# Autodesk Inventor assembly: SMALLER
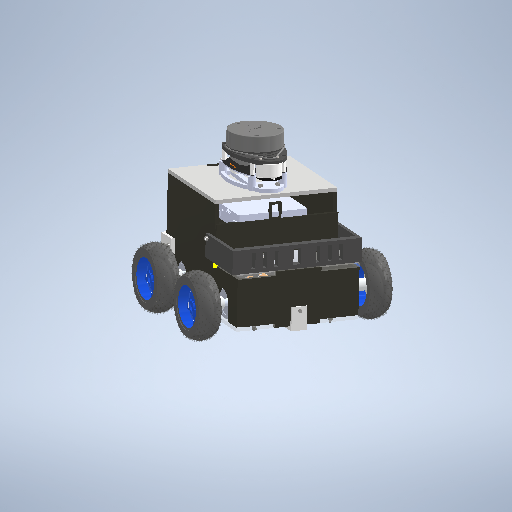
[picture p0: Inventor's stored thumbnail of the model, 512x512]
Saved by Autodesk Inventor 2025.3 (Build 293356030, 356C)
## iProperties
Created: 2026-06-30
Part Number: SMALLER
Document SubType Name: Assembly
Designer: user
Author: user
## Documents named in this file (14)
- C:\Docs\shcool\dojo\CAD_stuff\Final\SMALLER.iam
- C:\Docs\shcool\dojo\CAD_stuff\Final\WHEEL_BASE.iam
- C:\Docs\shcool\dojo\CAD_stuff\Final\back.ipt
- C:\Docs\shcool\dojo\CAD_stuff\Final\Fastener.ipt
- C:\Docs\shcool\dojo\CAD_stuff\Final\SIDE_1.ipt
- C:\Docs\shcool\dojo\CAD_stuff\Final\HOOD_1.ipt
- C:\Docs\shcool\dojo\CAD_stuff\Final\TOP_1.ipt
- C:\Docs\shcool\dojo\CAD_stuff\Final\FRONT_1.ipt
- C:\Docs\shcool\dojo\CAD_stuff\Final\COVER_1.ipt
- C:\Docs\shcool\dojo\CAD_stuff\Final\BONNET.ipt
- C:\Docs\shcool\dojo\CAD_stuff\Imports\assembled_lidar.iam
- C:\Docs\shcool\dojo\CAD_stuff\Design_3 - Copy\pi_internals\Complete_model.iam
- C:\Users\user\OneDrive\Documents\Inventor\Content Center Files\R2025\en-US\ISO 7040\DIEN EN ISO 7040 - M3.ipt
- C:\Users\user\OneDrive\Documents\Inventor\Content Center Files\R2025\en-US\ISO 4762(2)\ISO 4762 - M3 x 16ISO.ipt
## Components (48 placed, 13 different names)
1. WHEEL_BASE:1 [sub-assembly] — Mate:15, Mate:16, Mate:17, Mate:18, Mate:19, Insert:17
2. back:1 — Mate:5, Mate:6, Mate:7, Mate:8, Mate:9, Mate:12, Mate:14, Mate:15, Mate:21, Mate:23, Mate:24, Mate:25, Mate:26, Mate:27, Mate:28, Insert:25, Insert:29, Insert:30
3. SIDE_1:1 — Mate:5, Mate:6, Mate:7, Mate:13, Mate:32, Mate:33, Insert:20, Insert:31
4. SIDE_1:2 — Mate:8, Mate:9, Mate:16, Mate:20, Mate:22, Insert:28, Insert:34
5. Fastener:2 — Mate:20, Mate:21, Mate:22, Insert:7, Insert:8
6. Fastener:3 — Mate:12, Mate:13, Mate:14, Insert:9, Insert:10
7. Fastener:4 — Mate:17, Mate:18, Mate:19, Insert:3, Insert:4
8. HOOD_1:1 — Mate:23, Mate:24, Mate:30, Mate:31, Mate:47
9. TOP_1:1 — Mate:25, Mate:26, Mate:29, Insert:24, Mate:48, Insert:39, Insert:40, Insert:41, Insert:42
10. Fastener:5 — Mate:27, Mate:28, Mate:29, Insert:5, Insert:6
11. FRONT_1:1 — Mate:30, Mate:31, Mate:34, Mate:35, Mate:36
12. COVER_1:1 — Mate:32, Mate:33, Mate:42, Mate:43
13. Fastener:6 — Mate:34, Mate:35, Mate:36, Insert:1, Insert:2, Insert:18
14. BONNET:1 — Mate:47, Insert:32, Insert:33
15. Complete_model:1 [sub-assembly] — Mate:42, Mate:43
16. DIN EN ISO 7040 M3:1 — Insert:18
17. ISO 4762 M3 x 16:2 — Insert:4
18. ISO 4762 M3 x 16:3 — Insert:3
19. ISO 4762 M3 x 16:4 — Insert:1, Insert:27
20. ISO 4762 M3 x 16:5 — Insert:2
21. DIN EN ISO 7040 M3:2 — Insert:17
22. DIN EN ISO 7040 M3:3 — Insert:31
23. DIN EN ISO 7040 M3:4
24. DIN EN ISO 7040 M3:5 — Insert:20
25. ISO 4762 M3 x 16:6 — Insert:10
26. ISO 4762 M3 x 16:7 — Insert:9
27. ISO 4762 M3 x 16:8 — Insert:5
28. ISO 4762 M3 x 16:9 — Insert:8
29. ISO 4762 M3 x 16:10 — Insert:7
30. ISO 4762 M3 x 16:11 — Insert:6
31. DIN EN ISO 7040 M3:6 — Insert:27
32. DIN EN ISO 7040 M3:11 — Insert:24
33. DIN EN ISO 7040 M3:12 — Insert:25
34. DIN EN ISO 7040 M3:13 — Insert:28
35. DIN EN ISO 7040 M3:14 — Insert:29
36. DIN EN ISO 7040 M3:15 — Insert:30
37. DIN EN ISO 7040 M3:17 — Insert:34
38. ISO 4762 M3 x 16:16 — Insert:32
39. ISO 4762 M3 x 16:17 — Insert:33
40. assembled_lidar:1 [sub-assembly] — Mate:48, Insert:35, Insert:36, Insert:37, Insert:38
41. ISO 4762 M3 x 16:18 — Insert:38
42. DIN EN ISO 7040 M3:18 — Insert:39
43. ISO 4762 M3 x 16:19 — Insert:36
44. ISO 4762 M3 x 16:20 — Insert:35
45. ISO 4762 M3 x 16:21 — Insert:37
46. DIN EN ISO 7040 M3:19 — Insert:42
47. DIN EN ISO 7040 M3:20 — Insert:41
48. DIN EN ISO 7040 M3:21 — Insert:40
## Relationships (65: Mate 34, Insert 31)
- Mate:5: back:1 ↔ SIDE_1:1
- Mate:6: back:1 ↔ SIDE_1:1
- Mate:7: back:1 ↔ SIDE_1:1
- Mate:8: back:1 ↔ SIDE_1:2
- Mate:9: back:1 ↔ SIDE_1:2
- Mate:12: back:1 ↔ Fastener:3
- Mate:13: SIDE_1:1 ↔ Fastener:3
- Mate:14: back:1 ↔ Fastener:3
- Mate:15: WHEEL_BASE:1 ↔ back:1
- Mate:16: WHEEL_BASE:1 ↔ SIDE_1:2
- Mate:17: WHEEL_BASE:1 ↔ Fastener:4
- Mate:18: WHEEL_BASE:1 ↔ Fastener:4
- Mate:19: WHEEL_BASE:1 ↔ Fastener:4
- Mate:20: SIDE_1:2 ↔ Fastener:2
- Mate:21: back:1 ↔ Fastener:2
- Mate:22: SIDE_1:2 ↔ Fastener:2
- Mate:23: back:1 ↔ HOOD_1:1
- Mate:24: back:1 ↔ HOOD_1:1
- Mate:25: back:1 ↔ TOP_1:1
- Mate:26: back:1 ↔ TOP_1:1
- Mate:27: back:1 ↔ Fastener:5
- Mate:28: back:1 ↔ Fastener:5
- Mate:29: TOP_1:1 ↔ Fastener:5
- Mate:30: HOOD_1:1 ↔ FRONT_1:1
- Mate:31: HOOD_1:1 ↔ FRONT_1:1
- Mate:32: SIDE_1:1 ↔ COVER_1:1
- Mate:33: SIDE_1:1 ↔ COVER_1:1
- Mate:34: FRONT_1:1 ↔ Fastener:6
- Mate:35: FRONT_1:1 ↔ Fastener:6
- Mate:36: FRONT_1:1 ↔ Fastener:6
- Mate:42: COVER_1:1 ↔ Complete_model:1
- Mate:43: COVER_1:1 ↔ Complete_model:1
- Insert:1: Fastener:6 ↔ ISO 4762 M3 x 16:4
- Insert:2: Fastener:6 ↔ ISO 4762 M3 x 16:5
- Insert:3: Fastener:4 ↔ ISO 4762 M3 x 16:3
- Insert:4: Fastener:4 ↔ ISO 4762 M3 x 16:2
- Insert:5: Fastener:5 ↔ ISO 4762 M3 x 16:8
- Insert:6: Fastener:5 ↔ ISO 4762 M3 x 16:11
- Insert:7: Fastener:2 ↔ ISO 4762 M3 x 16:10
- Insert:8: Fastener:2 ↔ ISO 4762 M3 x 16:9
- Insert:9: Fastener:3 ↔ ISO 4762 M3 x 16:7
- Insert:10: Fastener:3 ↔ ISO 4762 M3 x 16:6
- Insert:17: WHEEL_BASE:1 ↔ DIN EN ISO 7040 M3:2
- Insert:18: Fastener:6 ↔ DIN EN ISO 7040 M3:1
- Insert:20: SIDE_1:1 ↔ DIN EN ISO 7040 M3:5
- Insert:24: TOP_1:1 ↔ DIN EN ISO 7040 M3:11
- Insert:25: back:1 ↔ DIN EN ISO 7040 M3:12
- Insert:27: ISO 4762 M3 x 16:4 ↔ DIN EN ISO 7040 M3:6
- Insert:28: SIDE_1:2 ↔ DIN EN ISO 7040 M3:13
- Insert:29: back:1 ↔ DIN EN ISO 7040 M3:14
- Insert:30: back:1 ↔ DIN EN ISO 7040 M3:15
- Insert:31: SIDE_1:1 ↔ DIN EN ISO 7040 M3:3
- Mate:47: HOOD_1:1 ↔ BONNET:1
- Insert:32: BONNET:1 ↔ ISO 4762 M3 x 16:16
- Insert:33: BONNET:1 ↔ ISO 4762 M3 x 16:17
- Insert:34: SIDE_1:2 ↔ DIN EN ISO 7040 M3:17
- Mate:48: TOP_1:1 ↔ assembled_lidar:1
- Insert:35: assembled_lidar:1 ↔ ISO 4762 M3 x 16:20
- Insert:36: assembled_lidar:1 ↔ ISO 4762 M3 x 16:19
- Insert:37: assembled_lidar:1 ↔ ISO 4762 M3 x 16:21
- Insert:38: assembled_lidar:1 ↔ ISO 4762 M3 x 16:18
- Insert:39: TOP_1:1 ↔ DIN EN ISO 7040 M3:18
- Insert:40: TOP_1:1 ↔ DIN EN ISO 7040 M3:21
- Insert:41: TOP_1:1 ↔ DIN EN ISO 7040 M3:20
- Insert:42: TOP_1:1 ↔ DIN EN ISO 7040 M3:19
